# Autodesk Inventor assembly: arm stop 48 degree 2 piece
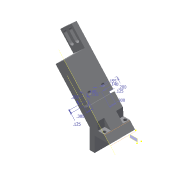
[picture p0: Inventor's stored thumbnail of the model, 180x180]
Saved by Autodesk Inventor 2018 (Build 220112000, 112)
## iProperties
Created: 2019-01-02
Part Number: arm stop 48 degree 2 piece
Document SubType Name: Assembly
Designer: ball
Author: ball
## Documents named in this file (3)
- C:\FTC\FTC8863CAD\2018Robot\arm stop 48 degree 2 piece.iam
- C:\FTC\FTC8863CAD\2018Robot\arm stop 48 degree top half.ipt
- C:\FTC\FTC8863CAD\2018Robot\arm stop 48 degree bottom half.ipt
## Components (2 placed, 2 different names)
1. arm stop 48 degree top half:1 — Mate:1, Flush:1
2. arm stop 48 degree bottom half:1 — Mate:1, Flush:1
## Relationships (2: Mate 1, Flush 1)
- Mate:1: arm stop 48 degree top half:1 ↔ arm stop 48 degree bottom half:1
- Flush:1: arm stop 48 degree top half:1 ↔ arm stop 48 degree bottom half:1
